# Autodesk Inventor assembly: Assembly_LED
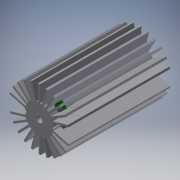
[picture p0: Inventor's stored thumbnail of the model, 180x180]
Saved by Autodesk Inventor 2018 (Build 220112000, 112)
## iProperties
Created: 2018-06-28
Part Number: Assembly_LED
Document SubType Name: Assembly
Designer: David
Author: David
## Documents named in this file (4)
- C:\Users\David\Documents\optoelectronics\CAD\LED\Assembly_LED.iam
- C:\Users\David\Documents\optoelectronics\CAD\LED\base.ipt
- C:\Users\David\Documents\optoelectronics\CAD\LED\front.ipt
- C:\Users\David\Documents\optoelectronics\CAD\LED\M850D2.ipt
## Components (3 placed, 3 different names)
1. base:1 — Mate:5, Mate:6, Flush:1, Mate:9
2. front:1 — Mate:5, Mate:6, Flush:1
3. M850D2:1 — Mate:9
## Relationships (4: Mate 3, Flush 1)
- Mate:5: base:1 ↔ front:1
- Mate:6: base:1 ↔ front:1
- Flush:1: base:1 ↔ front:1
- Mate:9: base:1 ↔ M850D2:1
